# Autodesk Inventor assembly: Assembly1
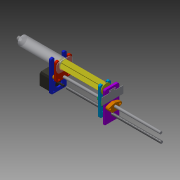
[picture p0: Inventor's stored thumbnail of the model, 180x180]
Saved by Autodesk Inventor 2015 SP1 (Build 190203100, 203)
## iProperties
Created: 2016-07-07
Part Number: Assembly1
Document SubType Name: Assembly
Designer: lustinga
Mass: 233.614 g
Surface Area: 1371.78 cm^2
Volume: 233.614 cm^3
Density: 1 g/cm^3
Author: lustinga
## Documents named in this file (15)
- Z:\Dropbox (HHMI)\JANELIA\Parkinsons Project\Syringe Pump\3D CAD\Syringe assembly.iam
- Z:\Dropbox (HHMI)\JANELIA\Parkinsons Project\Syringe Pump\3D CAD\motor mount.ipt
- Z:\Dropbox (HHMI)\JANELIA\Parkinsons Project\Syringe Pump\3D CAD\motor.ipt
- Z:\Dropbox (HHMI)\JANELIA\Parkinsons Project\Syringe Pump\3D CAD\syringe outer.ipt
- Z:\Dropbox (HHMI)\JANELIA\Parkinsons Project\Syringe Pump\3D CAD\syringe inner.ipt
- Z:\Dropbox (HHMI)\JANELIA\Parkinsons Project\Syringe Pump\3D CAD\8mm shaft.ipt
- Z:\Dropbox (HHMI)\JANELIA\Parkinsons Project\Syringe Pump\3D CAD\carriage.ipt
- Z:\Dropbox (HHMI)\JANELIA\Parkinsons Project\Syringe Pump\3D CAD\ACME rod.ipt
- Z:\Dropbox (HHMI)\JANELIA\Parkinsons Project\Syringe Pump\3D CAD\shaft support.ipt
- Z:\Dropbox (HHMI)\JANELIA\Parkinsons Project\Syringe Pump\3D CAD\linear bearing.ipt
- Z:\Dropbox (HHMI)\JANELIA\Parkinsons Project\Syringe Pump\3D CAD\end cap.ipt
- Z:\Dropbox (HHMI)\JANELIA\Parkinsons Project\Syringe Pump\3D CAD\acme nut.ipt
- Z:\Dropbox (HHMI)\JANELIA\Parkinsons Project\Syringe Pump\3D CAD\neck support.ipt
- Z:\Dropbox (HHMI)\JANELIA\Parkinsons Project\Syringe Pump\3D CAD\PCB.ipt
- Z:\Dropbox (HHMI)\JANELIA\Parkinsons Project\Syringe Pump\3D CAD\reed_switch.ipt
## Components (15 placed, 14 different names)
1. syringe inner:1 — Mate:13, Mate:112
2. syringe outer:1 — Mate:13, Mate:72, Mate:73, Flush:12
3. motor:1 — Mate:83, Mate:84, Flush:13, Mate:85, Mate:87, Flush:92, Flush:93, Flush:94
4. motor mount:1 — Mate:72, Flush:12, Mate:84, Flush:13, Mate:85, Mate:86, Flush:14, Mate:116, Mate:118, Mate:119
5. shaft support:1 — Mate:116, Mate:117, Mate:118, Mate:120, Mate:121, Mate:122
6. 8mm shaft:1 — Mate:77, Mate:86, Flush:14, Mate:106, Mate:115, Mate:117, Mate:126
7. ACME rod:1 — Mate:83, Mate:87, Mate:91, Mate:103, Mate:105
8. acme nut:1 — Mate:103, Mate:107, Mate:108, Mate:109
9. linear bearing:1 — Mate:77, Mate:111
10. carriage:2 — Mate:105, Mate:106, Mate:107, Mate:108, Mate:109, Mate:111, Mate:112, Mate:119
11. end cap:2 — Mate:91, Mate:115, Mate:123, Mate:124, Mate:125, Mate:127, Mate:128, Mate:129, Mate:130, Mate:131
12. shaft support:2 — Mate:126, Mate:127, Mate:128
13. neck support:1 — Mate:120, Mate:121, Mate:122, Mate:73
14. PCB:1 — Mate:123, Mate:124, Mate:125
15. reed_switch:1 — Mate:129, Mate:130, Mate:131
## Relationships (41: Mate 35, Flush 6)
- Mate:13: syringe inner:1 ↔ syringe outer:1
- Mate:72: syringe outer:1 ↔ motor mount:1
- Mate:73: syringe outer:1 ↔ neck support:1
- Flush:12: syringe outer:1 ↔ motor mount:1
- Mate:77: 8mm shaft:1 ↔ linear bearing:1
- Mate:83: motor:1 ↔ ACME rod:1
- Mate:84: motor:1 ↔ motor mount:1
- Flush:13: motor:1 ↔ motor mount:1
- Mate:85: motor:1 ↔ motor mount:1
- Mate:86: motor mount:1 ↔ 8mm shaft:1
- Mate:87 (10 mm): motor:1 ↔ ACME rod:1
- Flush:14: motor mount:1 ↔ 8mm shaft:1
- Flush:92: motor:1
- Flush:93: motor:1
- Flush:94: motor:1
- Mate:91: ACME rod:1 ↔ end cap:2
- Mate:103: ACME rod:1 ↔ acme nut:1
- Mate:105: ACME rod:1 ↔ carriage:2
- Mate:106: 8mm shaft:1 ↔ carriage:2
- Mate:107: acme nut:1 ↔ carriage:2
- Mate:108: acme nut:1 ↔ carriage:2
- Mate:109: acme nut:1 ↔ carriage:2
- Mate:111: linear bearing:1 ↔ carriage:2
- Mate:112: syringe inner:1 ↔ carriage:2
- Mate:115: 8mm shaft:1 ↔ end cap:2
- Mate:116: motor mount:1 ↔ shaft support:1
- Mate:117: shaft support:1 ↔ 8mm shaft:1
- Mate:118: motor mount:1 ↔ shaft support:1
- Mate:119 (40 mm): motor mount:1 ↔ carriage:2
- Mate:120: shaft support:1 ↔ neck support:1
- Mate:121: shaft support:1 ↔ neck support:1
- Mate:122: shaft support:1 ↔ neck support:1
- Mate:123: end cap:2 ↔ PCB:1
- Mate:124: end cap:2 ↔ PCB:1
- Mate:125: end cap:2 ↔ PCB:1
- Mate:126: 8mm shaft:1 ↔ shaft support:2
- Mate:127: end cap:2 ↔ shaft support:2
- Mate:128: end cap:2 ↔ shaft support:2
- Mate:129: end cap:2 ↔ reed_switch:1
- Mate:130: end cap:2 ↔ reed_switch:1
- Mate:131: end cap:2 ↔ reed_switch:1
